# Autodesk Inventor assembly: Motor Board w. Drivers
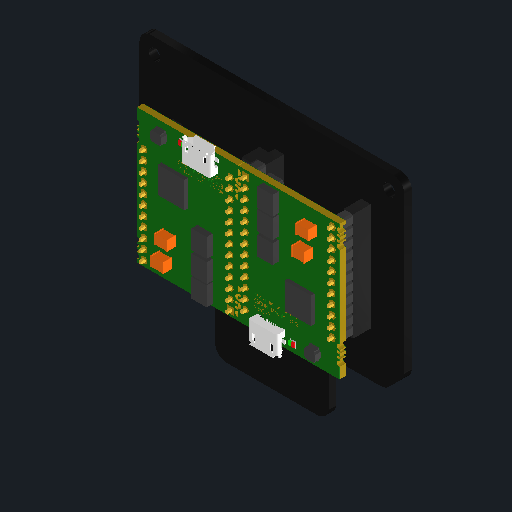
[picture p0: Inventor's stored thumbnail of the model, 512x512]
Saved by Autodesk Inventor 2026.1 (Build 301233020, 233B)
## iProperties
Created: 2026-04-03
Part Number: Motor Board w. Drivers
Document SubType Name: Assembly
Designer: Bahaa
Mass: 18.0608 g
Surface Area: 305.351 cm^2
Volume: 13.9205 cm^3
Density: 1.29742 g/cm^3
Author: Bahaa
## Documents named in this file (5)
- C:\Users\Bahaa\Nextcloud2\CAD\25-26\V2\Boards\Motor Board w. Drivers.iam
- C:\Users\Bahaa\Nextcloud2\CAD\25-26\V2\Boards\Motor Driver Board.ipt
- C:\Users\Bahaa\Nextcloud2\CAD\25-26\V2\Parts\466023_escon_module_24-2.ipt
- C:\Users\Bahaa\Nextcloud2\CAD\25-26\V2\Parts\11er Pin Header Female.ipt
- C:\Users\Bahaa\Nextcloud2\CAD\25-26\V2\Parts\13-Pin Header - Female - 2.54mm.ipt
## Components (7 placed, 4 different names)
1. Motor Driver Board:1 — Mate:3, Mate:6, Flush:12
2. 466023_escon_module_24-2:1 — Flush:1, Flush:2, Mate:1, Flush:3, Flush:4, Mate:2, Flush:10, Flush:11, Mate:7, Flush:12
3. 11er Pin Header Female:1 — Flush:3, Flush:4, Mate:2
4. 13-Pin Header - Female - 2.54mm:1 — Flush:1, Flush:2, Mate:1, Mate:3
5. 466023_escon_module_24-2:2 — Flush:10, Mate:7
6. 11er Pin Header Female:2
7. 13-Pin Header - Female - 2.54mm:2 — Mate:6
## Relationships (18: Flush 11, Mate 7)
- Flush:1: 466023_escon_module_24-2:1 ↔ 13-Pin Header - Female - 2.54mm:1
- Flush:2: 466023_escon_module_24-2:1 ↔ 13-Pin Header - Female - 2.54mm:1
- Mate:1: 466023_escon_module_24-2:1 ↔ 13-Pin Header - Female - 2.54mm:1
- Flush:3: 466023_escon_module_24-2:1 ↔ 11er Pin Header Female:1
- Flush:4: 466023_escon_module_24-2:1 ↔ 11er Pin Header Female:1
- Mate:2: 466023_escon_module_24-2:1 ↔ 11er Pin Header Female:1
- Mate:3: Motor Driver Board:1 ↔ 13-Pin Header - Female - 2.54mm:1
- [Flush]: 466023_escon_module_24-2:2 ↔ 13-Pin Header - Female - 2.54mm:2
- [Flush]: 466023_escon_module_24-2:2 ↔ 13-Pin Header - Female - 2.54mm:2
- [Mate]: 466023_escon_module_24-2:2 ↔ 13-Pin Header - Female - 2.54mm:2
- [Flush]: 466023_escon_module_24-2:2 ↔ 11er Pin Header Female:2
- [Flush]: 466023_escon_module_24-2:2 ↔ 11er Pin Header Female:2
- [Mate]: 466023_escon_module_24-2:2 ↔ 11er Pin Header Female:2
- Mate:6: Motor Driver Board:1 ↔ 13-Pin Header - Female - 2.54mm:2
- Flush:10: 466023_escon_module_24-2:1 ↔ 466023_escon_module_24-2:2
- Flush:11 (0.1 mm): 466023_escon_module_24-2:1
- Mate:7 (0.2 mm): 466023_escon_module_24-2:1 ↔ 466023_escon_module_24-2:2
- Flush:12 (5 mm): Motor Driver Board:1 ↔ 466023_escon_module_24-2:1
## Named parameters: d7_d0 = 0 mm, d8_d1 = 0 mm, d9_d2 = 0 mm, d10_d3 = 0 mm, d11_d4 = 0 mm, d12_d5 = 0 mm
